# Autodesk Inventor assembly: Assembly_Z_stage
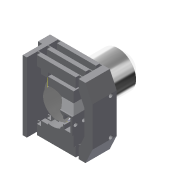
[picture p0: Inventor's stored thumbnail of the model, 180x180]
Saved by Autodesk Inventor 2019.4 (Build 234330000, 330)
## iProperties
Created: 2020-04-29
Part Number: Assembly_Z_stage
Document SubType Name: Assembly
Designer: diederichbenedict
Author: diederichbenedict
## Documents named in this file (3)
- C:\Users\diederichbenedict\Dropbox\Dokumente\Promotion\PROJECTS\STORMoChip\GITHUB\CAD\Nanoscopy-on-the-cheap\Workspace\Assembly_Z_stage.iam
- C:\Users\diederichbenedict\Dropbox\Dokumente\Promotion\PROJECTS\STORMoChip\GITHUB\CAD\Nanoscopy-on-the-cheap\Workspace\cellSTORM_v5_focussingunit_1.ipt
- C:\Users\diederichbenedict\Dropbox\Dokumente\Promotion\PROJECTS\STORMoChip\GITHUB\CAD\Nanoscopy-on-the-cheap\Workspace\00_Microscope_Objective.ipt
## Components (2 placed, 2 different names)
1. cellSTORM_v5_focussingunit_1:1 — Angle:2
2. 00_Microscope_Objective:1 — Angle:2
## Relationships (1: Angle 1)
- Angle:2 (0 deg): cellSTORM_v5_focussingunit_1:1 ↔ 00_Microscope_Objective:1
